# Autodesk Inventor assembly: Сборка2
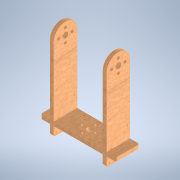
[picture p0: Inventor's stored thumbnail of the model, 180x180]
Saved by Autodesk Inventor 2020.1 (Build 241239000, 239)
## iProperties
Created: 2021-08-12
Part Number: Сборка2
Document SubType Name: Assembly
Designer: Ni3na
Author: Ni3na
## Documents named in this file (3)
- C:\Users\Ni3na\Documents\GitHub\avatar-kvantoriada\3D\Сборка2.iam
- C:\Users\Ni3na\Documents\GitHub\avatar-kvantoriada\3D\Деталь2.ipt
- C:\Users\Ni3na\Documents\GitHub\avatar-kvantoriada\3D\Деталь 3.ipt
## Components (3 placed, 2 different names)
1. Деталь2:1 — Жесткий:1, Жесткий:2
2. Деталь 3:1 — Жесткий:1
3. Деталь 3:2 — Жесткий:2
## Relationships (2: WeldJoint 2)
- Жесткий:1 [WeldJoint]: Деталь2:1 ↔ Деталь 3:1
- Жесткий:2 [WeldJoint]: Деталь2:1 ↔ Деталь 3:2
